# Autodesk Inventor assembly: Gripper_Assembly_SubAssembly
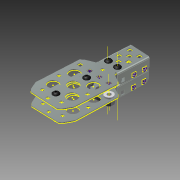
[picture p0: Inventor's stored thumbnail of the model, 180x180]
Saved by Autodesk Inventor 2013 (Build 170138000, 138)
## iProperties
Created: 2007-10-23
Part Number: Gripper_Assembly_SubAssembly
Document SubType Name: Assembly
Designer: Tyler
Author: Tyler
## Documents named in this file (7)
- C:\Data Folder\VEX 2012\VEX KOP Uploads\2013\Metric\Motion\Components\Gripper_Assembly_SubAssembly.iam
- C:\Data Folder\VEX 2012\VEX KOP Uploads\2013\Metric\Motion\Components\BEARING-FLAT.ipt
- C:\Data Folder\VEX 2012\VEX KOP Uploads\2013\Metric\Motion\Components\SCREW-832_SBS0832-0250ZB.ipt
- C:\Data Folder\VEX 2012\VEX KOP Uploads\2013\Metric\Motion\Components\BEAM-0500.ipt
- C:\Data Folder\VEX 2012\VEX KOP Uploads\2013\Metric\Motion\Components\BEARING-RIVET.ipt
- C:\Data Folder\VEX 2012\VEX KOP Uploads\2013\Metric\Motion\Components\WASHER-TEFLON.ipt
- C:\Data Folder\VEX 2012\VEX KOP Uploads\2013\Metric\Motion\Components\VEX Bracket.ipt
## Components (19 placed, 6 different names)
1. BEARING-FLAT — Mate:124, Mate:125, Mate:150, Mate:151, Mate:152
2. BEAM-0500 — Mate:32, Mate:38, Mate:104, Mate:120, Mate:121
3. SCREW-832_SBS0832-0250ZB — Mate:38, Mate:104, Mate:122
4. SCREW-832_SBS0832-0250ZB — Mate:32, Mate:118, Mate:119, Mate:120
5. BEARING-RIVET — Insert:11
6. WASHER-TEFLON — Insert:14
7. WASHER-TEFLON — Insert:13, Insert:14
8. BEARING-RIVET — Insert:12
9. VEX Bracket:1 — Mate:122, Insert:8, Mate:135, Angle:1, Mate:136, Angle:2, Mate:138, Mate:143, Mate:144, Mate:145, Mate:150, Mate:151, Mate:152, Insert:11, Insert:12, Insert:13
10. VEX Bracket:2 — Mate:118, Mate:119, Mate:121, Mate:124, Mate:125, Insert:9, Insert:10, Mate:141, Mate:146, Mate:147, Mate:149
11. SCREW-832_SBS0832-0250ZB:7 — Insert:8
12. SCREW-832_SBS0832-0250ZB:8 — Insert:9
13. BEAM-0500:4 — Insert:10
14. SCREW-832_SBS0832-0250ZB:9 — Mate:146, Mate:147, Mate:148
15. SCREW-832_SBS0832-0250ZB:10 — Mate:140, Mate:141
16. BEAM-0500:5 — Mate:148, Mate:149
17. BEAM-0500:6 — Mate:143
18. SCREW-832_SBS0832-0250ZB:11 — Mate:144, Mate:145
19. SCREW-832_SBS0832-0250ZB:12 — Mate:137, Mate:138, Mate:140
## Relationships (35: Mate 26, Insert 7, Angle 2)
- Mate:32: BEAM-0500 ↔ SCREW-832_SBS0832-0250ZB
- Mate:38: BEAM-0500 ↔ SCREW-832_SBS0832-0250ZB
- Mate:104: BEAM-0500 ↔ SCREW-832_SBS0832-0250ZB
- Mate:118: SCREW-832_SBS0832-0250ZB ↔ VEX Bracket:2
- Mate:119: SCREW-832_SBS0832-0250ZB ↔ VEX Bracket:2
- Mate:120: BEAM-0500 ↔ SCREW-832_SBS0832-0250ZB
- Mate:121: BEAM-0500 ↔ VEX Bracket:2
- Mate:122: SCREW-832_SBS0832-0250ZB ↔ VEX Bracket:1
- Mate:124: BEARING-FLAT ↔ VEX Bracket:2
- Mate:125: BEARING-FLAT ↔ VEX Bracket:2
- Insert:8: VEX Bracket:1 ↔ SCREW-832_SBS0832-0250ZB:7
- Insert:9: VEX Bracket:2 ↔ SCREW-832_SBS0832-0250ZB:8
- Insert:10: VEX Bracket:2 ↔ BEAM-0500:4
- Mate:135: VEX Bracket:1
- Angle:1 (0 deg): VEX Bracket:1
- Mate:136: VEX Bracket:1
- Angle:2 (0 deg): VEX Bracket:1
- Mate:137: SCREW-832_SBS0832-0250ZB:12
- Mate:138: VEX Bracket:1 ↔ SCREW-832_SBS0832-0250ZB:12
- Mate:140: SCREW-832_SBS0832-0250ZB:10 ↔ SCREW-832_SBS0832-0250ZB:12
- Mate:141: VEX Bracket:2 ↔ SCREW-832_SBS0832-0250ZB:10
- Mate:143: VEX Bracket:1 ↔ BEAM-0500:6
- Mate:144: VEX Bracket:1 ↔ SCREW-832_SBS0832-0250ZB:11
- Mate:145: VEX Bracket:1 ↔ SCREW-832_SBS0832-0250ZB:11
- Mate:146: VEX Bracket:2 ↔ SCREW-832_SBS0832-0250ZB:9
- Mate:147: VEX Bracket:2 ↔ SCREW-832_SBS0832-0250ZB:9
- Mate:148: SCREW-832_SBS0832-0250ZB:9 ↔ BEAM-0500:5
- Mate:149: VEX Bracket:2 ↔ BEAM-0500:5
- Mate:150: BEARING-FLAT ↔ VEX Bracket:1
- Mate:151: BEARING-FLAT ↔ VEX Bracket:1
- Mate:152: BEARING-FLAT ↔ VEX Bracket:1
- Insert:11: BEARING-RIVET ↔ VEX Bracket:1
- Insert:12: BEARING-RIVET ↔ VEX Bracket:1
- Insert:13: WASHER-TEFLON ↔ VEX Bracket:1
- Insert:14: WASHER-TEFLON
